# Autodesk Inventor assembly: L1 Gearbox Assembly
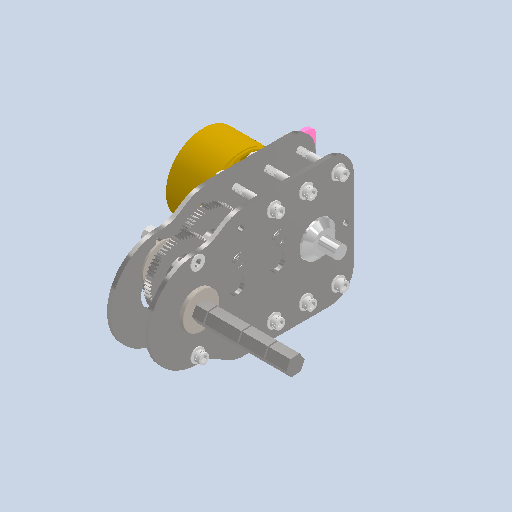
[picture p0: Inventor's stored thumbnail of the model, 512x512]
Saved by Autodesk Inventor 2025.1 (Build 291241020, 241B)
## iProperties
Created: 2023-02-14
Part Number: L1 Gearbox Assembly
Document SubType Name: Assembly
Designer: Dave
Mass: 913.46 g
Surface Area: 1660.69 cm^2
Volume: 243.163 cm^3
Density: 3.75658 g/cm^3
Author: Dave
## Documents named in this file (15)
- C:\Users\t205b\OneDrive\Documents\Github\BehrendURCMechanical\CAD\Chassis V3\CH3-L1SingleGearbox.iam
- C:\Users\t205b\OneDrive\Documents\Github\BehrendURCMechanical\CAD\Chassis V3\[Retired] GearBox\Final Gears and Assemblies\CH-1-01-20T_Drive Gear.ipt
- C:\Users\t205b\OneDrive\Documents\Github\BehrendURCMechanical\CAD\Chassis V3\[Retired] GearBox\Final Gears and Assemblies\CH-1-01-60T_Output.ipt
- C:\Users\t205b\OneDrive\Documents\Github\BehrendURCMechanical\CAD\Chassis V3\[Retired] GearBox\Final Gears and Assemblies\CH-1-01-20T_Idler.ipt
- C:\Users\t205b\OneDrive\Documents\Github\BehrendURCMechanical\CAD\Chassis V3\[Retired] GearBox\Final Gears and Assemblies\CH-1-01-60T_Idler.ipt
- C:\Users\t205b\OneDrive\Documents\Github\BehrendURCMechanical\CAD\Chassis [Retired]\GearBox\Drive Motor Shaft Coupler.ipt
- C:\Users\t205b\OneDrive\Documents\Github\BehrendURCMechanical\CAD\Chassis [Retired]\GearBox\Ch-1-01-0.5x4.5HexShaft.ipt
- C:\Users\t205b\OneDrive\Documents\Github\BehrendURCMechanical\CAD\Chassis [Retired]\GearBox\CH-1-01-0.25x1.875SmoothShaft.ipt
- C:\Users\t205b\OneDrive\Documents\Github\BehrendURCMechanical\CAD\Chassis [Retired]\GearBox\CH-1-01-0.5HexBearing.ipt
- C:\Users\t205b\OneDrive\Documents\Github\BehrendURCMechanical\CAD\Chassis [Retired]\GearBox\CH-1-01-0.25IDSmoothBoreBearing.ipt
- C:\Users\t205b\OneDrive\Documents\Github\BehrendURCMechanical\CAD\Chassis V3\DriveMotorAssem\DriveMotorAssem.iam
- C:\Users\t205b\OneDrive\Documents\Github\BehrendURCMechanical\CAD\Chassis V3\Hardware\91251A252_Black-Oxide Alloy Steel Socket Head Screw.ipt
- C:\Users\t205b\OneDrive\Documents\Github\BehrendURCMechanical\CAD\Chassis V3\Hardware\91831A011_18-8 Stainless Steel Nylon-Insert Locknut.ipt
- C:\Users\t205b\OneDrive\Documents\Github\BehrendURCMechanical\CAD\Chassis V3\Hardware\90107A011_316 Stainless Steel Washer.ipt
- C:\Users\t205b\OneDrive\Documents\Github\BehrendURCMechanical\CAD\Chassis V3\L1Plate.ipt
## Components (51 placed, 14 different names)
1. CH-1-01-20T_Drive Gear:1 — Insert:16
2. CH-1-01-60T_Output:1 — Mate:17, Flush:6
3. CH-1-01-20T_Idler:1 — Mate:21, Flush:5
4. CH-1-01-60T_Idler:1 — Mate:18, Mate:19, Mate:20, Flush:5
5. CH-1-01-20T_Idler:2 — Mate:19, Mate:22, Flush:6
6. CH-1-01-60T_Idler:2 — Mate:10, Mate:11
7. Drive Motor Shaft Coupler:1 — Insert:16, Mate:27, Mate:31, Mate:32
8. DriveMotorAssem:1 [sub-assembly] — Mate:27, Insert:59, Insert:60, Insert:61, Insert:66, Angle:2, Insert:67, Insert:68, Insert:69
9. Ch-1-01-0.5x4.5HexShaft:1 — Mate:8, Mate:9, Flush:8
10. CH-1-01-0.25x1.875SmoothShaft:1 — Insert:13
11. CH-1-01-0.25x1.875SmoothShaft:2 — Insert:12, Flush:4
12. CH-1-01-0.5HexBearing:1 — Mate:17, Flush:8, Mate:33
13. CH-1-01-0.5HexBearing:2 — Mate:8, Mate:9, Mate:29, Mate:30
14. CH-1-01-0.25IDSmoothBoreBearing:1 — Insert:12
15. CH-1-01-0.25IDSmoothBoreBearing:2 — Insert:13, Mate:11
16. CH-1-01-0.25IDSmoothBoreBearing:3 — Flush:4, Mate:18, Mate:20, Mate:22
17. CH-1-01-0.25IDSmoothBoreBearing:4 — Mate:10, Mate:21
18. 91251A252_Black-Oxide Alloy Steel Socket Head Screw:1 — Insert:75
19. 91831A011_18-8 Stainless Steel Nylon-Insert Locknut:1 — Insert:85
20. 91251A252_Black-Oxide Alloy Steel Socket Head Screw:2 — Insert:74
21. 91831A011_18-8 Stainless Steel Nylon-Insert Locknut:2 — Insert:84
22. 91251A252_Black-Oxide Alloy Steel Socket Head Screw:3 — Insert:73
23. 91831A011_18-8 Stainless Steel Nylon-Insert Locknut:3 — Insert:83
24. 91251A252_Black-Oxide Alloy Steel Socket Head Screw:4 — Insert:76
25. 91831A011_18-8 Stainless Steel Nylon-Insert Locknut:4 — Insert:82
26. 91251A252_Black-Oxide Alloy Steel Socket Head Screw:5 — Insert:72
27. 91831A011_18-8 Stainless Steel Nylon-Insert Locknut:5 — Insert:80
28. 91251A252_Black-Oxide Alloy Steel Socket Head Screw:6 — Insert:71
29. 91831A011_18-8 Stainless Steel Nylon-Insert Locknut:6 — Insert:79
30. 91251A252_Black-Oxide Alloy Steel Socket Head Screw:7 — Insert:70
31. 91831A011_18-8 Stainless Steel Nylon-Insert Locknut:7 — Insert:81
32. 91251A252_Black-Oxide Alloy Steel Socket Head Screw:8 — Insert:77
33. 91831A011_18-8 Stainless Steel Nylon-Insert Locknut:8 — Insert:78
34. 90107A011_316 Stainless Steel Washer:1 — Insert:61, Insert:82
35. 90107A011_316 Stainless Steel Washer:2 — Insert:75
36. 90107A011_316 Stainless Steel Washer:3 — Insert:74
37. 90107A011_316 Stainless Steel Washer:4 — Insert:60, Insert:83
38. 90107A011_316 Stainless Steel Washer:5 — Insert:73
39. 90107A011_316 Stainless Steel Washer:6 — Insert:59, Insert:84
40. 90107A011_316 Stainless Steel Washer:7 — Insert:53, Insert:76
41. 90107A011_316 Stainless Steel Washer:8 — Insert:51, Insert:85
42. 90107A011_316 Stainless Steel Washer:9 — Insert:57, Insert:77
43. 90107A011_316 Stainless Steel Washer:10 — Insert:55, Insert:78
44. 90107A011_316 Stainless Steel Washer:11 — Insert:70
45. 90107A011_316 Stainless Steel Washer:12 — Insert:67, Insert:79
46. 90107A011_316 Stainless Steel Washer:13 — Insert:71
47. 90107A011_316 Stainless Steel Washer:14 — Insert:68, Insert:80
48. 90107A011_316 Stainless Steel Washer:15 — Insert:72
49. 90107A011_316 Stainless Steel Washer:16 — Insert:69, Insert:81
50. L1Plate:1 — Mate:29, Insert:53, Insert:57, Mate:32
51. L1Plate:2 — Mate:30, Mate:31, Insert:51, Insert:55, Insert:66, Angle:2, Mate:33
## Relationships (51: Insert 30, Mate 16, Flush 4, Angle 1)
- Mate:8: Ch-1-01-0.5x4.5HexShaft:1 ↔ CH-1-01-0.5HexBearing:2
- Mate:9: Ch-1-01-0.5x4.5HexShaft:1 ↔ CH-1-01-0.5HexBearing:2
- Insert:12: CH-1-01-0.25x1.875SmoothShaft:2 ↔ CH-1-01-0.25IDSmoothBoreBearing:1
- Insert:13: CH-1-01-0.25x1.875SmoothShaft:1 ↔ CH-1-01-0.25IDSmoothBoreBearing:2
- Mate:10: CH-1-01-60T_Idler:2 ↔ CH-1-01-0.25IDSmoothBoreBearing:4
- Mate:11: CH-1-01-60T_Idler:2 ↔ CH-1-01-0.25IDSmoothBoreBearing:2
- Flush:4: CH-1-01-0.25x1.875SmoothShaft:2 ↔ CH-1-01-0.25IDSmoothBoreBearing:3
- Mate:17: CH-1-01-60T_Output:1 ↔ CH-1-01-0.5HexBearing:1
- Mate:18: CH-1-01-60T_Idler:1 ↔ CH-1-01-0.25IDSmoothBoreBearing:3
- Mate:19: CH-1-01-60T_Idler:1 ↔ CH-1-01-20T_Idler:2
- Mate:20: CH-1-01-60T_Idler:1 ↔ CH-1-01-0.25IDSmoothBoreBearing:3
- Mate:21: CH-1-01-20T_Idler:1 ↔ CH-1-01-0.25IDSmoothBoreBearing:4
- Flush:5: CH-1-01-20T_Idler:1 ↔ CH-1-01-60T_Idler:1
- Mate:22: CH-1-01-20T_Idler:2 ↔ CH-1-01-0.25IDSmoothBoreBearing:3
- Flush:6: CH-1-01-60T_Output:1 ↔ CH-1-01-20T_Idler:2
- Flush:8: Ch-1-01-0.5x4.5HexShaft:1 ↔ CH-1-01-0.5HexBearing:1
- Insert:16: CH-1-01-20T_Drive Gear:1 ↔ Drive Motor Shaft Coupler:1
- Mate:27: Drive Motor Shaft Coupler:1 ↔ DriveMotorAssem:1
- Mate:29: CH-1-01-0.5HexBearing:2 ↔ L1Plate:1
- Mate:30: CH-1-01-0.5HexBearing:2 ↔ L1Plate:2
- Mate:31: Drive Motor Shaft Coupler:1 ↔ L1Plate:2
- Insert:51: 90107A011_316 Stainless Steel Washer:8 ↔ L1Plate:2
- Insert:53: 90107A011_316 Stainless Steel Washer:7 ↔ L1Plate:1
- Insert:55: 90107A011_316 Stainless Steel Washer:10 ↔ L1Plate:2
- Insert:57: 90107A011_316 Stainless Steel Washer:9 ↔ L1Plate:1
- Insert:59: DriveMotorAssem:1 ↔ 90107A011_316 Stainless Steel Washer:6
- Insert:60: DriveMotorAssem:1 ↔ 90107A011_316 Stainless Steel Washer:4
- Insert:61: DriveMotorAssem:1 ↔ 90107A011_316 Stainless Steel Washer:1
- Insert:66: DriveMotorAssem:1 ↔ L1Plate:2
- Angle:2 (0 deg): DriveMotorAssem:1 ↔ L1Plate:2
- Insert:67: DriveMotorAssem:1 ↔ 90107A011_316 Stainless Steel Washer:12
- Insert:68: DriveMotorAssem:1 ↔ 90107A011_316 Stainless Steel Washer:14
- Insert:69: DriveMotorAssem:1 ↔ 90107A011_316 Stainless Steel Washer:16
- Mate:32: Drive Motor Shaft Coupler:1 ↔ L1Plate:1
- Insert:70: 91251A252_Black-Oxide Alloy Steel Socket Head Screw:7 ↔ 90107A011_316 Stainless Steel Washer:11
- Insert:71: 91251A252_Black-Oxide Alloy Steel Socket Head Screw:6 ↔ 90107A011_316 Stainless Steel Washer:13
- Insert:72: 91251A252_Black-Oxide Alloy Steel Socket Head Screw:5 ↔ 90107A011_316 Stainless Steel Washer:15
- Insert:73: 91251A252_Black-Oxide Alloy Steel Socket Head Screw:3 ↔ 90107A011_316 Stainless Steel Washer:5
- Insert:74: 91251A252_Black-Oxide Alloy Steel Socket Head Screw:2 ↔ 90107A011_316 Stainless Steel Washer:3
- Insert:75: 91251A252_Black-Oxide Alloy Steel Socket Head Screw:1 ↔ 90107A011_316 Stainless Steel Washer:2
- Insert:76: 91251A252_Black-Oxide Alloy Steel Socket Head Screw:4 ↔ 90107A011_316 Stainless Steel Washer:7
- Insert:77: 91251A252_Black-Oxide Alloy Steel Socket Head Screw:8 ↔ 90107A011_316 Stainless Steel Washer:9
- Insert:78: 91831A011_18-8 Stainless Steel Nylon-Insert Locknut:8 ↔ 90107A011_316 Stainless Steel Washer:10
- Insert:79: 91831A011_18-8 Stainless Steel Nylon-Insert Locknut:6 ↔ 90107A011_316 Stainless Steel Washer:12
- Insert:80: 91831A011_18-8 Stainless Steel Nylon-Insert Locknut:5 ↔ 90107A011_316 Stainless Steel Washer:14
- Insert:81: 91831A011_18-8 Stainless Steel Nylon-Insert Locknut:7 ↔ 90107A011_316 Stainless Steel Washer:16
- Insert:82: 91831A011_18-8 Stainless Steel Nylon-Insert Locknut:4 ↔ 90107A011_316 Stainless Steel Washer:1
- Insert:83: 91831A011_18-8 Stainless Steel Nylon-Insert Locknut:3 ↔ 90107A011_316 Stainless Steel Washer:4
- Insert:84: 91831A011_18-8 Stainless Steel Nylon-Insert Locknut:2 ↔ 90107A011_316 Stainless Steel Washer:6
- Insert:85: 91831A011_18-8 Stainless Steel Nylon-Insert Locknut:1 ↔ 90107A011_316 Stainless Steel Washer:8
- Mate:33: CH-1-01-0.5HexBearing:1 ↔ L1Plate:2
